# Autodesk Inventor assembly: B_Legs0
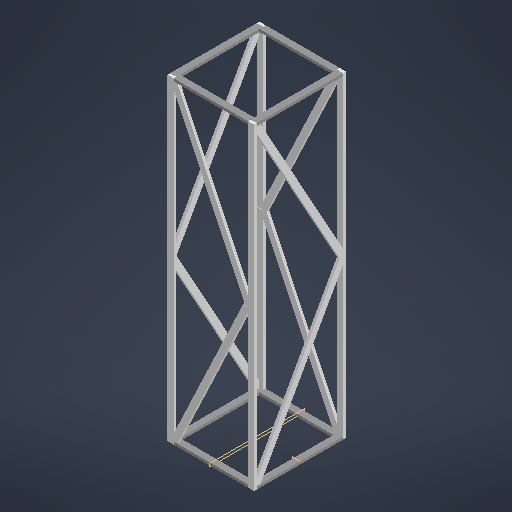
[picture p0: Inventor's stored thumbnail of the model, 512x512]
Saved by Autodesk Inventor 2026 (Build 300175000, 175)
## iProperties
Created: 2024-09-19
Part Number: B_Legs0
Document SubType Name: Assembly
Designer: User
Author: User
## Documents named in this file (8)
- C:\Users\trott\Documents\UofSC-ASME-Tiger-Burn-Design-2025\CAD\Legs\Front Leg\F_Leg.iam
- C:\Users\trott\Documents\UofSC-ASME-Tiger-Burn-Design-2025\CAD\Legs\Front Leg\2x4x42.ipt
- C:\Users\trott\Documents\UofSC-ASME-Tiger-Burn-Design-2025\CAD\Legs\Front Leg\2x4x48.ipt
- C:\Users\trott\Documents\UofSC-ASME-Tiger-Burn-Design-2025\CAD\Legs\Front Leg\2x4x176.ipt
- C:\Users\trott\Documents\UofSC-ASME-Tiger-Burn-Design-2025\CAD\Legs\Front Leg\S_2x4x98.925.ipt
- C:\Users\trott\Documents\UofSC-ASME-Tiger-Burn-Design-2025\CAD\Legs\Front Leg\S_2x4x102.079.ipt
- C:\Users\trott\Documents\UofSC-ASME-Tiger-Burn-Design-2025\CAD\Legs\Front Leg\S_2x4x99.417.ipt
- C:\Users\trott\Documents\UofSC-ASME-Tiger-Burn-Design-2025\CAD\Legs\Front Leg\S_2x4x95.725.ipt
## Components (20 placed, 7 different names)
1. S_2x4x98.925:1 — Mate:23, Flush:39
2. S_2x4x102.079:1 — Mate:25, Flush:42
3. S_2x4x102.079:2 — Mate:26, Flush:43
4. S_2x4x98.925:2 — Mate:27, Flush:44
5. S_2x4x99.417:1 — Mate:28, Flush:45
6. S_2x4x99.417:2 — Mate:29, Mate:30, Flush:46
7. S_2x4x95.725:1 — Mate:31, Mate:32, Flush:47
8. S_2x4x95.725:2 — Mate:33, Mate:34, Flush:48
9. 2x4x176:2 — Mate:24, Flush:40, Flush:41, Mate:29, Flush:46, Mate:31, Flush:47
10. 2x4x176:1 — Flush:27, Mate:18, Flush:28, Mate:19, Flush:30, Flush:39, Flush:43
11. 2x4x176:3 — Flush:42
12. 2x4x176:4 — Flush:45, Mate:33, Flush:48
13. 2x4x42:5 — Flush:27, Mate:18, Flush:28, Flush:29, Mate:34
14. 2x4x42:6 — Mate:32
15. 2x4x42:7 — Mate:28
16. 2x4x42:8 — Mate:30
17. 2x4x48:5 — Flush:29, Mate:19, Flush:30, Flush:31, Flush:34, Mate:23, Mate:24, Flush:40, Flush:41
18. 2x4x48:6 — Mate:26
19. 2x4x48:7 — Mate:27, Flush:44
20. 2x4x48:8 — Mate:25
## Component patterns: (2 elements, first: 2x4x176:2 + 2x4x176:1), (4 elements, first: 2x4x42:5), (4 elements, first: 2x4x48:5)
## Relationships (30: Flush 16, Mate 14)
- Flush:27: 2x4x176:1 ↔ 2x4x42:5
- Mate:18: 2x4x176:1 ↔ 2x4x42:5
- Flush:28: 2x4x176:1 ↔ 2x4x42:5
- Flush:29: 2x4x42:5 ↔ 2x4x48:5
- Mate:19: 2x4x176:1 ↔ 2x4x48:5
- Flush:30: 2x4x176:1 ↔ 2x4x48:5
- Flush:31 (520.7 mm): 2x4x48:5
- Flush:34 (-609.6 mm): 2x4x48:5
- Mate:23: S_2x4x98.925:1 ↔ 2x4x48:5
- Flush:39: S_2x4x98.925:1 ↔ 2x4x176:1
- Mate:24: 2x4x176:2 ↔ 2x4x48:5
- Flush:40: 2x4x176:2 ↔ 2x4x48:5
- Flush:41: 2x4x176:2 ↔ 2x4x48:5
- Mate:25: S_2x4x102.079:1 ↔ 2x4x48:8
- Flush:42: S_2x4x102.079:1 ↔ 2x4x176:3
- Mate:26: S_2x4x102.079:2 ↔ 2x4x48:6
- Flush:43: S_2x4x102.079:2 ↔ 2x4x176:1
- Mate:27: S_2x4x98.925:2 ↔ 2x4x48:7
- Flush:44: S_2x4x98.925:2 ↔ 2x4x48:7
- Mate:28: S_2x4x99.417:1 ↔ 2x4x42:7
- Flush:45: S_2x4x99.417:1 ↔ 2x4x176:4
- Mate:29: S_2x4x99.417:2 ↔ 2x4x176:2
- Mate:30: S_2x4x99.417:2 ↔ 2x4x42:8
- Flush:46: S_2x4x99.417:2 ↔ 2x4x176:2
- Mate:31: S_2x4x95.725:1 ↔ 2x4x176:2
- Mate:32: S_2x4x95.725:1 ↔ 2x4x42:6
- Flush:47: S_2x4x95.725:1 ↔ 2x4x176:2
- Mate:33: S_2x4x95.725:2 ↔ 2x4x176:4
- Mate:34: S_2x4x95.725:2 ↔ 2x4x42:5
- Flush:48: S_2x4x95.725:2 ↔ 2x4x176:4
